# Autodesk Inventor assembly: atxInterface
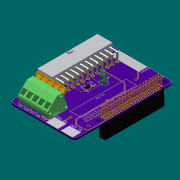
[picture p0: Inventor's stored thumbnail of the model, 180x180]
Saved by Autodesk Inventor 2016 SP1 (Build 200210100, 210)
## iProperties
Created: 2016-04-06
Part Number: atxInterface
Document SubType Name: Assembly
Designer: Sawaiz
Author: Sawaiz
## Documents named in this file (9)
- C:\Users\Sawaiz\OneDrive\projects\atxInterface\cad\atxInterface.iam
- C:\Users\Sawaiz\OneDrive\projects\atxInterface\cad\electronics\SOT23-3.ipt
- C:\Users\Sawaiz\OneDrive\projects\atxInterface\cad\electronics\chipResistor\chipResistor-0805.ipt
- C:\Users\Sawaiz\OneDrive\projects\atxInterface\cad\electronics\chipResistor.ipt
- C:\Users\Sawaiz\OneDrive\projects\atxInterface\cad\electronics\5mmLed.ipt
- C:\Users\Sawaiz\OneDrive\projects\atxInterface\cad\connectors\molexMiniFitJr24.ipt
- C:\Users\Sawaiz\OneDrive\projects\atxInterface\cad\atxInterfacePcb.ipt
- C:\Users\Sawaiz\OneDrive\projects\atxInterface\cad\connectors\terminalBlock.ipt
- C:\Users\Sawaiz\OneDrive\projects\atxInterface\cad\connectors\2.54Header\piExtraTall\2x20ExtraTallHeader.iam
## Components (14 placed, 7 different names)
1. SOT23-3:1 — Angle:4, Flush:3, Flush:4, Angle:7, Angle:8, Angle:10
2. chipResistor-0805:1 — Flush:1, Flush:2, Flush:3, Mate:2, Angle:10
3. chipResistor-0805:2 — Flush:1, Angle:4, Angle:8, Angle:9, Flush:10
4. chipResistor-0805:3 — Flush:2, Angle:6, Angle:7
5. 5mmLed:1 — Flush:4, Angle:9
6. molexMiniFitJr24:1 — Mate:1, Angle:5, Flush:9
7. atxInterfacePcb:1 — Mate:1, Angle:5, Mate:2, Angle:6, Mate:3, Angle:11, Angle:12
8. terminalBlock:1 — Mate:3, Angle:11, Mate:4, Flush:5, Flush:6, Mate:8, Mate:9
9. terminalBlock:2 — Mate:4, Mate:5, Flush:5, Mate:8, Flush:9, Flush:10, Mate:12
10. terminalBlock:3 — Mate:5, Mate:6, Flush:6, Flush:7, Mate:9, Mate:10
11. terminalBlock:4 — Mate:6, Mate:7, Flush:7, Flush:8, Mate:10, Mate:11
12. terminalBlock:5 — Mate:7, Flush:8, Mate:11
13. atxInterfacePcb:2 — Mate:12, Mate:13
14. 2x20ExtraTallHeader:1 [sub-assembly] — Mate:13, Angle:12
## Relationships (32: Mate 13, Flush 10, Angle 9)
- Flush:1: chipResistor-0805:1 ↔ chipResistor-0805:2
- Flush:2: chipResistor-0805:1 ↔ chipResistor-0805:3
- Angle:4 (0 deg): SOT23-3:1 ↔ chipResistor-0805:2
- Mate:1: molexMiniFitJr24:1 ↔ atxInterfacePcb:1
- Angle:5 (0 deg): molexMiniFitJr24:1 ↔ atxInterfacePcb:1
- Flush:3: SOT23-3:1 ↔ chipResistor-0805:1
- Flush:4: SOT23-3:1 ↔ 5mmLed:1
- Mate:2: chipResistor-0805:1 ↔ atxInterfacePcb:1
- Angle:6 (0 deg): chipResistor-0805:3 ↔ atxInterfacePcb:1
- Angle:7 (0 deg): SOT23-3:1 ↔ chipResistor-0805:3
- Angle:8 (0 deg): SOT23-3:1 ↔ chipResistor-0805:2
- Angle:9 (0 deg): chipResistor-0805:2 ↔ 5mmLed:1
- Angle:10 (0 deg): SOT23-3:1 ↔ chipResistor-0805:1
- Mate:3: atxInterfacePcb:1 ↔ terminalBlock:1
- Angle:11 (0 deg): atxInterfacePcb:1 ↔ terminalBlock:1
- Mate:4: terminalBlock:1 ↔ terminalBlock:2
- Mate:5: terminalBlock:2 ↔ terminalBlock:3
- Mate:6: terminalBlock:3 ↔ terminalBlock:4
- Mate:7: terminalBlock:4 ↔ terminalBlock:5
- Flush:5: terminalBlock:1 ↔ terminalBlock:2
- Flush:6: terminalBlock:1 ↔ terminalBlock:3
- Flush:7: terminalBlock:3 ↔ terminalBlock:4
- Flush:8: terminalBlock:4 ↔ terminalBlock:5
- Mate:8: terminalBlock:1 ↔ terminalBlock:2
- Mate:9: terminalBlock:1 ↔ terminalBlock:3
- Mate:10: terminalBlock:3 ↔ terminalBlock:4
- Mate:11: terminalBlock:4 ↔ terminalBlock:5
- Flush:9: molexMiniFitJr24:1 ↔ terminalBlock:2
- Flush:10: chipResistor-0805:2 ↔ terminalBlock:2
- Mate:12: terminalBlock:2 ↔ atxInterfacePcb:2
- Mate:13: atxInterfacePcb:2 ↔ 2x20ExtraTallHeader:1
- Angle:12 (0 deg): atxInterfacePcb:1 ↔ 2x20ExtraTallHeader:1
